# Autodesk Inventor assembly: Quatro V6 Silent System
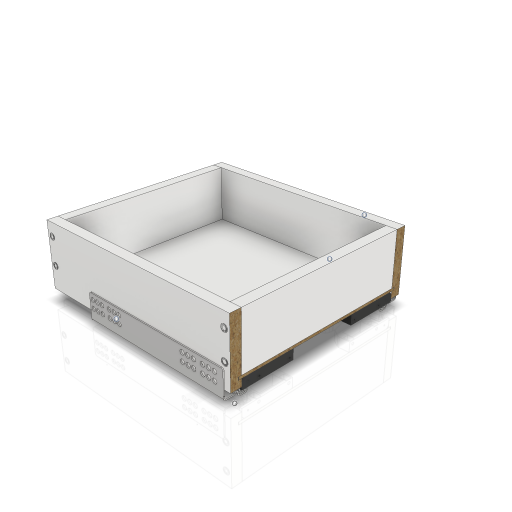
[picture p0: Inventor's stored thumbnail of the model, 512x512]
Saved by Autodesk Inventor 2024 (Build 280153000, 153)
## iProperties
Category: Drawer
RuleStatus: InUse
Created: 2014-06-26
Part Number: Quatro V6 Silent System
Document SubType Name: Assembly
Designer: SauliusD
Description: Hettich Quatro V6 Silent System Drawer
AfterAnyParamChange0: Drawer_Configuration
Author: SauliusD
## Documents named in this file (15)
- C:\W4INV 2024 Design\iBOX LIBRARY\Drawers\Hettich Quadro\Quatro V6 Silent System.iam
- C:\W4INV 2024 Design\iBOX LIBRARY\Drawers\Hettich Quadro\Parts\Left Drawer side.ipt
- C:\W4INV 2024 Design\iBOX LIBRARY\Drawers\Hettich Quadro\Parts\Right Drawer Side.ipt
- C:\W4INV 2024 Design\iBOX LIBRARY\Drawers\Hettich Quadro\Parts\Drawer Bottom.ipt
- C:\W4INV 2024 Design\iBOX LIBRARY\Drawers\Hettich Quadro\Parts\Drawer Front.ipt
- C:\W4INV 2024 Design\iBOX LIBRARY\Drawers\Hettich Quadro\Parts\Drawer Back.ipt
- C:\W4INV 2024 Design\iBOX LIBRARY\Drawers\Hettich Quadro\Subs\Left Runner.iam
- C:\W4INV 2024 Design\iBOX LIBRARY\Drawers\Hettich Quadro\Subs\Right Runner.iam
- C:\W4INV 2024 Design\iBOX LIBRARY\Drawers\Hettich Quadro\Parts\Left Sillet.ipt
- C:\W4INV 2024 Design\iBOX LIBRARY\Drawers\Hettich Quadro\Parts\Right Sillent.ipt
- C:\W4INV 2024 Design\iBOX LIBRARY\Drawers\Hettich Quadro\Parts\Right Catcher.ipt
- C:\W4INV 2024 Design\iBOX LIBRARY\Drawers\Hettich Quadro\Parts\Left Cather.ipt
- C:\W4INV 2024 Design\iBOX LIBRARY\Drawers\Hettich Quadro\Parts\Quatro V6 Silent System.ipt
- C:\W4INV 2024 Design\_LIBRARY\Fixed joints\Confirmat\CONFIRMAT\Confirmat L50 NB T16 PB T 16.ipt
- C:\W4INV 2024 Design\LIBRARY\Fixed joints\Confirmat\CONFIRMAT.ipt
## Components (20 placed, 13 different names)
1. @Skeleton — Flush:3, Flush:4, Flush:5
2. Left Drawer side:1 — Mate:10, Nestled Board Plane:1, Nestled Board Plane:3, Nestled Board Plane:5, Nestled Board Plane:7
3. Right Drawer Side:1 — Mate:8, Nestled Board Plane:2, Nestled Board Plane:4, Nestled Board Plane:6, Nestled Board Plane:8
4. Drawer Bottom:1 — Mate:7, Mate:9
5. Drawer Front:1 — Flush:1, Flush:2, Flush:6, Flush:7, Pillar Board Side Plane:3, Pillar Board Side Plane:4, Pillar Board Side Plane:7, Pillar Board Side Plane:8
6. Drawer Back:1 — Pillar Board Side Plane:1, Pillar Board Side Plane:2, Pillar Board Side Plane:5, Pillar Board Side Plane:6
7. Left Runner:1 [sub-assembly] — Mate:1, Mate:2, Mate:3
8. Right Runner:1 [sub-assembly] — Mate:4, Mate:5, Mate:6
9. Left Sillet:1 — Mate:1, Mate:2, Mate:3
10. Right Sillent:1 — Mate:4, Mate:5, Mate:6
11. Right Catcher:2 — Mate:7, Flush:1, Mate:8
12. Left Cather:1 — Mate:9, Flush:2, Mate:10
13. Confirmat L50 NB T16 PB T 16:2 — Axis Plane:1, Pillar Board Side Plane:1, Nestled Board Plane:1
14. Confirmat L50 NB T16 PB T 16:3 — Axis Plane:2, Pillar Board Side Plane:2, Nestled Board Plane:2
15. Confirmat L50 NB T16 PB T 16:4 — Axis Plane:3, Pillar Board Side Plane:3, Nestled Board Plane:3
16. Confirmat L50 NB T16 PB T 16:5 — Axis Plane:4, Pillar Board Side Plane:4, Nestled Board Plane:4
17. Confirmat L50 NB T16 PB T 16:6 — Axis Plane:5, Pillar Board Side Plane:5, Nestled Board Plane:5
18. Confirmat L50 NB T16 PB T 16:7 — Axis Plane:6, Pillar Board Side Plane:6, Nestled Board Plane:6
19. Confirmat L50 NB T16 PB T 16:8 — Axis Plane:7, Pillar Board Side Plane:7, Nestled Board Plane:7
20. Confirmat L50 NB T16 PB T 16:9 — Axis Plane:8, Pillar Board Side Plane:8, Nestled Board Plane:8
## Relationships (41: Mate 26, Flush 15)
- Mate:1: Left Runner:1 ↔ Left Sillet:1
- Mate:2: Left Runner:1 ↔ Left Sillet:1
- Mate:3: Left Runner:1 ↔ Left Sillet:1
- Mate:4: Right Runner:1 ↔ Right Sillent:1
- Mate:5: Right Runner:1 ↔ Right Sillent:1
- Mate:6: Right Runner:1 ↔ Right Sillent:1
- Mate:7: Drawer Bottom:1 ↔ Right Catcher:2
- Flush:1: Drawer Front:1 ↔ Right Catcher:2
- Mate:8: Right Drawer Side:1 ↔ Right Catcher:2
- Mate:9: Drawer Bottom:1 ↔ Left Cather:1
- Flush:2: Drawer Front:1 ↔ Left Cather:1
- Mate:10: Left Drawer side:1 ↔ Left Cather:1
- Flush:3: @Skeleton
- Flush:4: @Skeleton
- Flush:5: @Skeleton
- Flush:6 (-20 mm): Drawer Front:1
- Flush:7 (-20 mm): Drawer Front:1
- Axis Plane:1 [Mate]: Confirmat L50 NB T16 PB T 16:2
- Pillar Board Side Plane:1 [Mate] (-8 mm): Drawer Back:1 ↔ Confirmat L50 NB T16 PB T 16:2
- Nestled Board Plane:1 [Flush]: Left Drawer side:1 ↔ Confirmat L50 NB T16 PB T 16:2
- Axis Plane:2 [Mate]: Confirmat L50 NB T16 PB T 16:3
- Pillar Board Side Plane:2 [Mate] (-8 mm): Drawer Back:1 ↔ Confirmat L50 NB T16 PB T 16:3
- Nestled Board Plane:2 [Flush]: Right Drawer Side:1 ↔ Confirmat L50 NB T16 PB T 16:3
- Axis Plane:3 [Mate]: Confirmat L50 NB T16 PB T 16:4
- Pillar Board Side Plane:3 [Mate] (-8 mm): Drawer Front:1 ↔ Confirmat L50 NB T16 PB T 16:4
- Nestled Board Plane:3 [Flush]: Left Drawer side:1 ↔ Confirmat L50 NB T16 PB T 16:4
- Axis Plane:4 [Mate]: Confirmat L50 NB T16 PB T 16:5
- Pillar Board Side Plane:4 [Mate] (-8 mm): Drawer Front:1 ↔ Confirmat L50 NB T16 PB T 16:5
- Nestled Board Plane:4 [Flush]: Right Drawer Side:1 ↔ Confirmat L50 NB T16 PB T 16:5
- Axis Plane:5 [Mate]: Confirmat L50 NB T16 PB T 16:6
- Pillar Board Side Plane:5 [Mate] (-8 mm): Drawer Back:1 ↔ Confirmat L50 NB T16 PB T 16:6
- Nestled Board Plane:5 [Flush]: Left Drawer side:1 ↔ Confirmat L50 NB T16 PB T 16:6
- Axis Plane:6 [Mate]: Confirmat L50 NB T16 PB T 16:7
- Pillar Board Side Plane:6 [Mate] (-8 mm): Drawer Back:1 ↔ Confirmat L50 NB T16 PB T 16:7
- Nestled Board Plane:6 [Flush]: Right Drawer Side:1 ↔ Confirmat L50 NB T16 PB T 16:7
- Axis Plane:7 [Mate]: Confirmat L50 NB T16 PB T 16:8
- Pillar Board Side Plane:7 [Mate] (-8 mm): Drawer Front:1 ↔ Confirmat L50 NB T16 PB T 16:8
- Nestled Board Plane:7 [Flush]: Left Drawer side:1 ↔ Confirmat L50 NB T16 PB T 16:8
- Axis Plane:8 [Mate]: Confirmat L50 NB T16 PB T 16:9
- Pillar Board Side Plane:8 [Mate] (-8 mm): Drawer Front:1 ↔ Confirmat L50 NB T16 PB T 16:9
- Nestled Board Plane:8 [Flush]: Right Drawer Side:1 ↔ Confirmat L50 NB T16 PB T 16:9
## Named parameters: ConfirmatOffset1 = -20 mm, ConfirmatOffset2 = -20 mm, Drawer_Height = 79.75 mm, Whole_Drawer_Height = 110 mm, Distance_from_bottom = 0 mm, Inlet = 0 mm, RearSpace = 5 mm
